# Autodesk Inventor assembly: UBG-Schuss
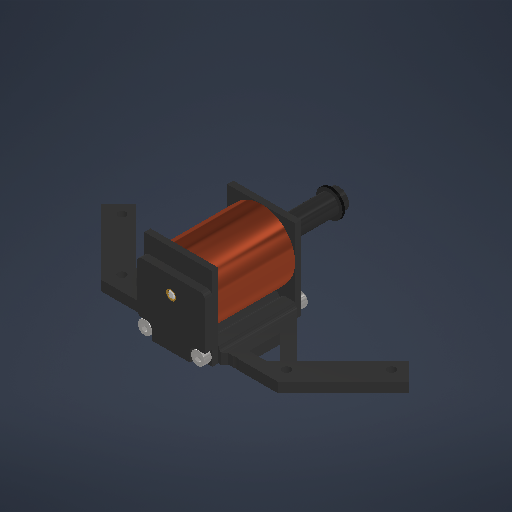
[picture p0: Inventor's stored thumbnail of the model, 512x512]
Saved by Autodesk Inventor 2025.2 (Build 292293000, 293)
## iProperties
Created: 2025-03-27
Part Number: UBG-Schuss
Document SubType Name: Assembly
Designer: Faabs
Author: Faabs
## Documents named in this file (8)
- C:\Users\Faabs\Desktop\TeamFaabs-CAD v2023\UBG\Schuss\UBG-Schuss.iam
- C:\Users\Faabs\Desktop\TeamFaabs-CAD v2023\UBG\Schuss\Schusshalterung\Schusshalterung\Schusshalterung.ipt
- C:\Users\Faabs\Desktop\TeamFaabs-CAD v2023\Verbindungselemente\Inventor\M3 Schmelzgewinde\M3 Schmelzgewinde\M3 Schmelzgewinde.ipt
- C:\Users\Faabs\Desktop\TeamFaabs-CAD v2023\UBG\Schuss\Schusskoerper\Schusskoerper\Schusskoerper.ipt
- C:\Users\Faabs\Desktop\TeamFaabs-CAD v2023\UBG\Schuss\Spulenkoerper\Spulenkoerper\Spulenkoerper.ipt
- C:\Users\Faabs\Desktop\TeamFaabs-CAD v2023\UBG\Schuss\Tauchkern\Tauchkern\Tauchkern.ipt
- C:\Users\Faabs\Desktop\TeamFaabs-CAD v2023\UBG\Schuss\Schussplatte\Schussplatte\Schussplatte.ipt
- C:\Users\Faabs\Desktop\TeamFaabs-CAD v2023\Verbindungselemente\Inventor\DIN 912\DIN 912 - M3 x 0,5 x 6 x 4,75.ipt
## Components (14 placed, 7 different names)
1. Schusshalterung:1 — Passend:1, Passend:2, Passend:3, Passend:4, Passend:5, Passend:6, Passend:7, Fluchtend:1, Fluchtend:2, Fluchtend:3, Fluchtend:4, Passend:10
2. Schusskoerper:1 — Passend:8, Passend:9, Passend:10, Passend:11, Passend:12, Passend:13, Winkel:1, Passend:16, Einfügen:1, Einfügen:2, Einfügen:3, Einfügen:4
3. Spulenkoerper:1 — Passend:11, Passend:12
4. Tauchkern:1 — Passend:13, Passend:15, Fluchtend:6
5. Schussplatte:1 — Passend:14, Fluchtend:5, Fluchtend:6, Winkel:1, Passend:16
6. M3 Schmelzgewinde:1 — Passend:2, Fluchtend:1
7. M3 Schmelzgewinde:2 — Passend:1, Fluchtend:2, Passend:8
8. M3 Schmelzgewinde:3 — Passend:4, Fluchtend:4, Passend:9
9. M3 Schmelzgewinde:4 — Passend:3, Fluchtend:3
10. M3 Schmelzgewinde:5 — Passend:14, Fluchtend:5, Passend:15
11. DIN 912 - ersetzt durch DIN EN ISO 4762 M3 x 6:1 — Einfügen:2
12. DIN 912 - ersetzt durch DIN EN ISO 4762 M3 x 6:2 — Einfügen:1
13. DIN 912 - ersetzt durch DIN EN ISO 4762 M3 x 6:3 — Einfügen:3
14. DIN 912 - ersetzt durch DIN EN ISO 4762 M3 x 6:4 — Einfügen:4
## Relationships (27: Mate 16, Flush 6, Insert 4, Angle 1)
- Passend:1 [Mate]: Schusshalterung:1 ↔ M3 Schmelzgewinde:2
- Passend:2 [Mate]: Schusshalterung:1 ↔ M3 Schmelzgewinde:1
- Passend:3 [Mate]: Schusshalterung:1 ↔ M3 Schmelzgewinde:4
- Passend:4 [Mate]: Schusshalterung:1 ↔ M3 Schmelzgewinde:3
- Passend:5 [Mate]: Schusshalterung:1
- Passend:6 [Mate]: Schusshalterung:1
- Passend:7 [Mate]: Schusshalterung:1
- Fluchtend:1 [Flush] (0.1 mm): Schusshalterung:1 ↔ M3 Schmelzgewinde:1
- Fluchtend:2 [Flush] (0.1 mm): Schusshalterung:1 ↔ M3 Schmelzgewinde:2
- Fluchtend:3 [Flush] (0.1 mm): Schusshalterung:1 ↔ M3 Schmelzgewinde:4
- Fluchtend:4 [Flush] (0.1 mm): Schusshalterung:1 ↔ M3 Schmelzgewinde:3
- Passend:8 [Mate]: Schusskoerper:1 ↔ M3 Schmelzgewinde:2
- Passend:9 [Mate]: Schusskoerper:1 ↔ M3 Schmelzgewinde:3
- Passend:10 [Mate]: Schusshalterung:1 ↔ Schusskoerper:1
- Passend:11 [Mate]: Schusskoerper:1 ↔ Spulenkoerper:1
- Passend:12 [Mate]: Schusskoerper:1 ↔ Spulenkoerper:1
- Passend:13 [Mate]: Schusskoerper:1 ↔ Tauchkern:1
- Passend:14 [Mate]: Schussplatte:1 ↔ M3 Schmelzgewinde:5
- Fluchtend:5 [Flush] (0.1 mm): Schussplatte:1 ↔ M3 Schmelzgewinde:5
- Passend:15 [Mate]: Tauchkern:1 ↔ M3 Schmelzgewinde:5
- Fluchtend:6 [Flush]: Tauchkern:1 ↔ Schussplatte:1
- Winkel:1 [Angle] (0 deg): Schusskoerper:1 ↔ Schussplatte:1
- Passend:16 [Mate]: Schusskoerper:1 ↔ Schussplatte:1
- Einfügen:1 [Insert]: Schusskoerper:1 ↔ DIN 912 - ersetzt durch DIN EN ISO 4762 M3 x 6:2
- Einfügen:2 [Insert]: Schusskoerper:1 ↔ DIN 912 - ersetzt durch DIN EN ISO 4762 M3 x 6:1
- Einfügen:3 [Insert]: Schusskoerper:1 ↔ DIN 912 - ersetzt durch DIN EN ISO 4762 M3 x 6:3
- Einfügen:4 [Insert]: Schusskoerper:1 ↔ DIN 912 - ersetzt durch DIN EN ISO 4762 M3 x 6:4
